# Autodesk Inventor assembly: MVPV1
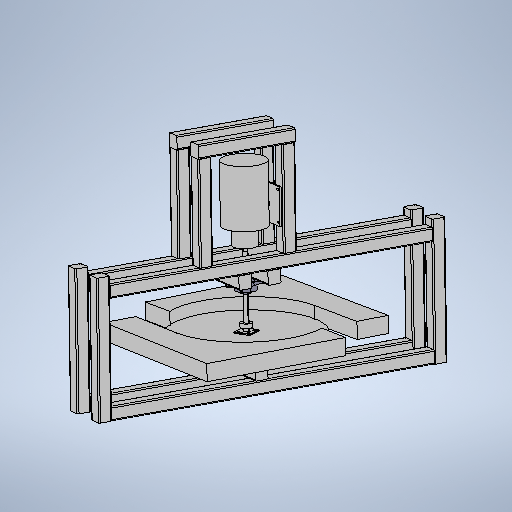
[picture p0: Inventor's stored thumbnail of the model, 512x512]
Saved by Autodesk Inventor 2025.1 (Build 291241000, 241)
## iProperties
Created: 2025-10-12
Part Number: MVPV1
Document SubType Name: Assembly
Designer: jonas
Author: jonas
## Documents named in this file (13)
- C:\Users\jonas\Documents\Studium\Master\3.Semester\StudentProject\SpinLauncher\drawings\MVPV1.iam
- C:\Users\jonas\Documents\Studium\Master\3.Semester\StudentProject\SpinLauncher\drawings\MotorV1.ipt
- C:\Users\jonas\Documents\Studium\Master\3.Semester\StudentProject\SpinLauncher\drawings\Item4040MotorVerticalV1.ipt
- C:\Users\jonas\Documents\Studium\Master\3.Semester\StudentProject\SpinLauncher\drawings\Item4040MotorHorizontalV1.ipt
- C:\Users\jonas\Documents\Studium\Master\3.Semester\StudentProject\SpinLauncher\drawings\Item4040RotorHorizontalV1.ipt
- C:\Users\jonas\Documents\Studium\Master\3.Semester\StudentProject\SpinLauncher\drawings\Item4040RotorVerticalV1.ipt
- C:\Users\jonas\Documents\Studium\Master\3.Semester\StudentProject\SpinLauncher\drawings\FlanschV1.ipt
- C:\Users\jonas\Documents\Studium\Master\3.Semester\StudentProject\SpinLauncher\drawings\RotorDiskV1.ipt
- C:\Users\jonas\Documents\Studium\Master\3.Semester\StudentProject\SpinLauncher\drawings\FlanschKugellager15mm\7508860.iam
- C:\Users\jonas\Documents\Studium\Master\3.Semester\StudentProject\SpinLauncher\drawings\Item4040BearingHolder.ipt
- C:\Users\jonas\Documents\Studium\Master\3.Semester\StudentProject\SpinLauncher\drawings\ShaftNut300mmV1.ipt
- C:\Users\jonas\Documents\Studium\Master\3.Semester\StudentProject\SpinLauncher\drawings\ShaftManschette15mmV1.ipt
- C:\Users\jonas\Documents\Studium\Master\3.Semester\StudentProject\SpinLauncher\drawings\WoodBoundaryV1.ipt
## Components (27 placed, 12 different names)
1. MotorV1:1 — Mate:1, Mate:2, Flush:1, Flush:2, Mate:17, Mate:18, Mate:24, Mate:30, Mate:31, Mate:38, Mate:39
2. Item4040MotorVerticalV1:1 — Mate:1, Flush:1, Flush:5, Mate:4, Flush:6, Mate:8, Flush:13
3. Item4040MotorVerticalV1:2 — Mate:2, Flush:2, Mate:3, Flush:3, Flush:4, Mate:7, Flush:11
4. Item4040MotorHorizontalV1:1 — Flush:5, Mate:4, Flush:6, Mate:6, Flush:9, Flush:10, Flush:26
5. Item4040MotorHorizontalV1:2 — Mate:3, Flush:3, Flush:4, Mate:5, Flush:7, Flush:8, Flush:26
6. Item4040MotorVerticalV1:3 — Mate:6, Flush:9, Flush:10, Flush:14
7. Item4040MotorVerticalV1:4 — Mate:5, Flush:7, Flush:8, Flush:12
8. Item4040RotorHorizontalV1:1 — Mate:7, Flush:11, Flush:12, Mate:9, Mate:11, Flush:15, Flush:17, Mate:21, Flush:29, Flush:30
9. Item4040RotorHorizontalV1:2 — Mate:8, Flush:13, Flush:14, Mate:10, Mate:12, Flush:16, Flush:18, Mate:22
10. Item4040RotorHorizontalV1:3 — Mate:14, Flush:19, Flush:22, Flush:24, Mate:19
11. Item4040RotorHorizontalV1:4 — Mate:13, Flush:20, Flush:21, Flush:23, Flush:28
12. Item4040RotorVerticalV1:1 — Mate:10, Flush:18, Flush:24
13. Item4040RotorVerticalV1:2 — Mate:9, Flush:17, Flush:23
14. Item4040RotorVerticalV1:3 — Mate:12, Flush:16, Mate:14, Flush:19, Flush:22, Flush:25, Flush:27
15. Item4040RotorVerticalV1:4 — Mate:11, Flush:15, Mate:13, Flush:20, Flush:21, Flush:25, Flush:27
16. FlanschV1:1 — Mate:15, Mate:16, Flush:31, Mate:35
17. RotorDiskV1:1 — Mate:15, Mate:16, Mate:17, Mate:36
18. 7508860:1 [sub-assembly] — Mate:18, Mate:20, Mate:28, Mate:29, Mate:37
19. Item4040BearingHolder:1 — Mate:19, Flush:28, Mate:20, Mate:28, Mate:29, Mate:32
20. Item4040BearingHolder:2 — Mate:22, Flush:30, Mate:26, Mate:27
21. Item4040BearingHolder:3 — Mate:21, Flush:29, Mate:23, Mate:25, Mate:26
22. 7508860:2 [sub-assembly] — Mate:23, Mate:24, Mate:25, Mate:27
23. ShaftNut300mmV1:1 — Mate:30, Mate:31, Mate:32, Flush:31, Mate:33, Mate:34
24. ShaftManschette15mmV1:1 — Mate:33, Mate:35
25. ShaftManschette15mmV1:2 — Mate:34, Mate:36, Mate:37
26. WoodBoundaryV1:1 — Mate:38
27. WoodBoundaryV1:2 — Mate:39
## Relationships (70: Mate 39, Flush 31)
- Mate:1: MotorV1:1 ↔ Item4040MotorVerticalV1:1
- Mate:2: MotorV1:1 ↔ Item4040MotorVerticalV1:2
- Flush:1 (-10 mm): MotorV1:1 ↔ Item4040MotorVerticalV1:1
- Flush:2 (10 mm): MotorV1:1 ↔ Item4040MotorVerticalV1:2
- Mate:3: Item4040MotorVerticalV1:2 ↔ Item4040MotorHorizontalV1:2
- Flush:3: Item4040MotorVerticalV1:2 ↔ Item4040MotorHorizontalV1:2
- Flush:4: Item4040MotorVerticalV1:2 ↔ Item4040MotorHorizontalV1:2
- Flush:5: Item4040MotorVerticalV1:1 ↔ Item4040MotorHorizontalV1:1
- Mate:4: Item4040MotorVerticalV1:1 ↔ Item4040MotorHorizontalV1:1
- Flush:6: Item4040MotorVerticalV1:1 ↔ Item4040MotorHorizontalV1:1
- Mate:5: Item4040MotorHorizontalV1:2 ↔ Item4040MotorVerticalV1:4
- Flush:7: Item4040MotorHorizontalV1:2 ↔ Item4040MotorVerticalV1:4
- Flush:8: Item4040MotorHorizontalV1:2 ↔ Item4040MotorVerticalV1:4
- Mate:6: Item4040MotorHorizontalV1:1 ↔ Item4040MotorVerticalV1:3
- Flush:9: Item4040MotorHorizontalV1:1 ↔ Item4040MotorVerticalV1:3
- Flush:10: Item4040MotorHorizontalV1:1 ↔ Item4040MotorVerticalV1:3
- Mate:7: Item4040MotorVerticalV1:2 ↔ Item4040RotorHorizontalV1:1
- Flush:11: Item4040MotorVerticalV1:2 ↔ Item4040RotorHorizontalV1:1
- Flush:12: Item4040MotorVerticalV1:4 ↔ Item4040RotorHorizontalV1:1
- Mate:8: Item4040MotorVerticalV1:1 ↔ Item4040RotorHorizontalV1:2
- Flush:13: Item4040MotorVerticalV1:1 ↔ Item4040RotorHorizontalV1:2
- Flush:14: Item4040MotorVerticalV1:3 ↔ Item4040RotorHorizontalV1:2
- Mate:9: Item4040RotorHorizontalV1:1 ↔ Item4040RotorVerticalV1:2
- Mate:10: Item4040RotorHorizontalV1:2 ↔ Item4040RotorVerticalV1:1
- Mate:11: Item4040RotorHorizontalV1:1 ↔ Item4040RotorVerticalV1:4
- Mate:12: Item4040RotorHorizontalV1:2 ↔ Item4040RotorVerticalV1:3
- Flush:15: Item4040RotorHorizontalV1:1 ↔ Item4040RotorVerticalV1:4
- Flush:16: Item4040RotorHorizontalV1:2 ↔ Item4040RotorVerticalV1:3
- Flush:17: Item4040RotorHorizontalV1:1 ↔ Item4040RotorVerticalV1:2
- Flush:18: Item4040RotorHorizontalV1:2 ↔ Item4040RotorVerticalV1:1
- Mate:13: Item4040RotorHorizontalV1:4 ↔ Item4040RotorVerticalV1:4
- Mate:14: Item4040RotorHorizontalV1:3 ↔ Item4040RotorVerticalV1:3
- Flush:19: Item4040RotorHorizontalV1:3 ↔ Item4040RotorVerticalV1:3
- Flush:20: Item4040RotorHorizontalV1:4 ↔ Item4040RotorVerticalV1:4
- Flush:21: Item4040RotorHorizontalV1:4 ↔ Item4040RotorVerticalV1:4
- Flush:22: Item4040RotorHorizontalV1:3 ↔ Item4040RotorVerticalV1:3
- Flush:23: Item4040RotorHorizontalV1:4 ↔ Item4040RotorVerticalV1:2
- Flush:24: Item4040RotorHorizontalV1:3 ↔ Item4040RotorVerticalV1:1
- Flush:25: Item4040RotorVerticalV1:3 ↔ Item4040RotorVerticalV1:4
- Flush:26: Item4040MotorHorizontalV1:1 ↔ Item4040MotorHorizontalV1:2
- Flush:27: Item4040RotorVerticalV1:3 ↔ Item4040RotorVerticalV1:4
- Mate:15: FlanschV1:1 ↔ RotorDiskV1:1
- Mate:16: FlanschV1:1 ↔ RotorDiskV1:1
- Mate:17: MotorV1:1 ↔ RotorDiskV1:1
- Mate:18: MotorV1:1 ↔ 7508860:1
- Mate:19: Item4040RotorHorizontalV1:3 ↔ Item4040BearingHolder:1
- Flush:28: Item4040RotorHorizontalV1:4 ↔ Item4040BearingHolder:1
- Mate:20: 7508860:1 ↔ Item4040BearingHolder:1
- Mate:21: Item4040RotorHorizontalV1:1 ↔ Item4040BearingHolder:3
- Mate:22: Item4040RotorHorizontalV1:2 ↔ Item4040BearingHolder:2
- Flush:29: Item4040RotorHorizontalV1:1 ↔ Item4040BearingHolder:3
- Flush:30: Item4040RotorHorizontalV1:1 ↔ Item4040BearingHolder:2
- Mate:23: Item4040BearingHolder:3 ↔ 7508860:2
- Mate:24: MotorV1:1 ↔ 7508860:2
- Mate:25 (-20 mm): Item4040BearingHolder:3 ↔ 7508860:2
- Mate:26 (-130 mm): Item4040BearingHolder:2 ↔ Item4040BearingHolder:3
- Mate:27 (-20 mm): Item4040BearingHolder:2 ↔ 7508860:2
- Mate:28 (-20 mm): 7508860:1 ↔ Item4040BearingHolder:1
- Mate:29 (-20 mm): 7508860:1 ↔ Item4040BearingHolder:1
- Mate:30: MotorV1:1 ↔ ShaftNut300mmV1:1
- Mate:31: MotorV1:1 ↔ ShaftNut300mmV1:1
- Mate:32: Item4040BearingHolder:1 ↔ ShaftNut300mmV1:1
- Flush:31: FlanschV1:1 ↔ ShaftNut300mmV1:1
- Mate:33: ShaftNut300mmV1:1 ↔ ShaftManschette15mmV1:1
- Mate:34: ShaftNut300mmV1:1 ↔ ShaftManschette15mmV1:2
- Mate:35 (10 mm): FlanschV1:1 ↔ ShaftManschette15mmV1:1
- Mate:36: RotorDiskV1:1 ↔ ShaftManschette15mmV1:2
- Mate:37 (10 mm): 7508860:1 ↔ ShaftManschette15mmV1:2
- Mate:38: MotorV1:1 ↔ WoodBoundaryV1:1
- Mate:39: MotorV1:1 ↔ WoodBoundaryV1:2
